# Autodesk Inventor assembly: 本体
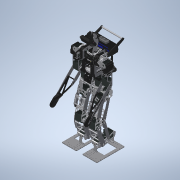
[picture p0: Inventor's stored thumbnail of the model, 180x180]
Saved by Autodesk Inventor 2020 (Build 240168000, 168)
## iProperties
Created: 2016-05-03
Part Number: 本体
Document SubType Name: Assembly
Designer: hiroaki
Mass: 3980.04 g
Surface Area: 11124 cm^2
Volume: 2032.65 cm^3
Density: 1.95805 g/cm^3
Author: hiroaki
## Documents named in this file (4)
- C:\Users\ito 017\Documents\GitHub\OpenPlatform\mechanism\OpenPlatform_ver3_0\本体.iam
- C:\Users\ito 017\Documents\GitHub\OpenPlatform\mechanism\OpenPlatform_ver3_0\上半身.iam
- C:\Users\ito 017\Documents\GitHub\OpenPlatform\mechanism\OpenPlatform_ver3_0\下半身_6.iam
- C:\Users\ito 017\Documents\GitHub\OpenPlatform\mechanism\OpenPlatform_ver3_0\下半身_6_MIR.iam
## Components (3 placed, 3 different names)
1. 上半身:1 [sub-assembly] — 挿入:1, 角度:1, 挿入:2, 角度:2, 角度:3
2. 下半身_6:1 [sub-assembly] — 挿入:1, 角度:1, 角度:3
3. 下半身_6_MIR:1 [sub-assembly] — 挿入:2, 角度:2
## Relationships (5: Angle 3, Insert 2)
- 挿入:1 [Insert]: 上半身:1 ↔ 下半身_6:1
- 角度:1 [Angle] (0 deg): 上半身:1 ↔ 下半身_6:1
- 挿入:2 [Insert]: 上半身:1 ↔ 下半身_6_MIR:1
- 角度:2 [Angle] (0 deg): 上半身:1 ↔ 下半身_6_MIR:1
- 角度:3 [Angle] (30 deg): 上半身:1 ↔ 下半身_6:1
